# Autodesk Inventor assembly: Assembly1
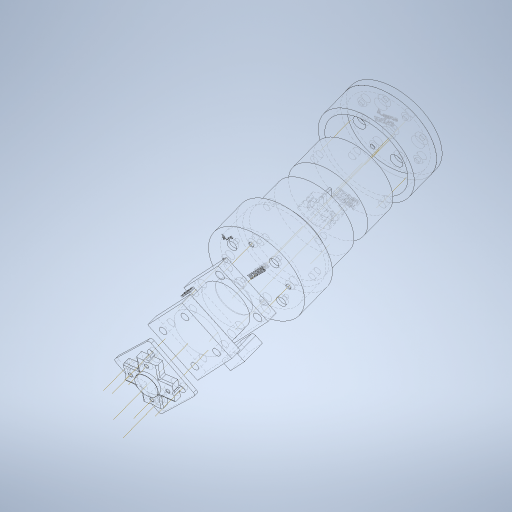
[picture p0: Inventor's stored thumbnail of the model, 512x512]
Saved by Autodesk Inventor 2024 (Build 280153000, 153)
## iProperties
Created: 2024-08-06
Part Number: Assembly1
Document SubType Name: Assembly
Designer: maint
Author: maint
## Documents named in this file (8)
- G:\3dprintings\Assembly1.iam
- G:\3dprintings\adapter_final2.ipt
- G:\3dprintings\adaptor_spine_transducer_names.ipt
- G:\3dprintings\adaptor_spine_base_names.ipt
- C:\Users\maint\Downloads\91292A770_18-8 Stainless Steel Socket Head Screw\91292A770_18-8 Stainless Steel Socket Head Screw.iam
- C:\Users\maint\Downloads\91263A913_Zinc-Plated Alloy Steel Hex Drive Flat Head Screw\91263A913_Zinc-Plated Alloy Steel Hex Drive Flat Head Screw.iam
- G:\3dprintings\spine.ipt
- G:\3dprintings\sensor_AMTI.ipt
## Components (17 placed, 7 different names)
1. adapter_final2:2 — Flush:2, Mate:3, Mate:5, Mate:9, Mate:11, Mate:14, Mate:16, Mate:20, Mate:21, Mate:24
2. adaptor_spine_transducer_names:1 — Flush:1, Flush:2, Mate:29, Mate:30, Mate:32, Mate:33, Mate:34, Mate:43, Mate:52
3. adaptor_spine_base_names:1 — Flush:1, Mate:26, Mate:45, Mate:46, Mate:47, Mate:48, Mate:57, Mate:58
4. 91292A770_18-8 Stainless Steel Socket Head Screw:1 [sub-assembly] — Mate:12
5. 91292A770_18-8 Stainless Steel Socket Head Screw:2 [sub-assembly] — Mate:2
6. 91292A770_18-8 Stainless Steel Socket Head Screw:3 [sub-assembly] — Mate:8, Mate:10
7. 91292A770_18-8 Stainless Steel Socket Head Screw:4 [sub-assembly] — Mate:6, Mate:7
8. 91263A913_Zinc-Plated Alloy Steel Hex Drive Flat Head Screw:1 [sub-assembly] — Mate:13, Mate:15
9. 91263A913_Zinc-Plated Alloy Steel Hex Drive Flat Head Screw:2 [sub-assembly] — Mate:17
10. 91263A913_Zinc-Plated Alloy Steel Hex Drive Flat Head Screw:3 [sub-assembly] — Mate:19
11. 91263A913_Zinc-Plated Alloy Steel Hex Drive Flat Head Screw:4 [sub-assembly] — Mate:18
12. 91292A770_18-8 Stainless Steel Socket Head Screw:5 [sub-assembly] — Mate:31
13. 91292A770_18-8 Stainless Steel Socket Head Screw:6 [sub-assembly] — Mate:36, Mate:37
14. 91292A770_18-8 Stainless Steel Socket Head Screw:7 [sub-assembly] — Mate:38
15. 91292A770_18-8 Stainless Steel Socket Head Screw:8 [sub-assembly] — Mate:40, Mate:41
16. spine:1 — Mate:42, Mate:43, Mate:44, Mate:49, Mate:50, Mate:57
17. sensor_AMTI:1 — Mate:51, Mate:54, Mate:55
## Relationships (57: Mate 55, Flush 2)
- Flush:1 (-203.2 mm): adaptor_spine_transducer_names:1 ↔ adaptor_spine_base_names:1
- Flush:2 (203.2 mm): adapter_final2:2 ↔ adaptor_spine_transducer_names:1
- Mate:2: 91292A770_18-8 Stainless Steel Socket Head Screw:2
- Mate:3: adapter_final2:2
- Mate:4
- Mate:5: adapter_final2:2
- Mate:6: 91292A770_18-8 Stainless Steel Socket Head Screw:4
- Mate:7: 91292A770_18-8 Stainless Steel Socket Head Screw:4
- Mate:8: 91292A770_18-8 Stainless Steel Socket Head Screw:3
- Mate:9: adapter_final2:2
- Mate:10: 91292A770_18-8 Stainless Steel Socket Head Screw:3
- Mate:11: adapter_final2:2
- Mate:12: 91292A770_18-8 Stainless Steel Socket Head Screw:1
- Mate:13: 91263A913_Zinc-Plated Alloy Steel Hex Drive Flat Head Screw:1
- Mate:14: adapter_final2:2
- Mate:15: 91263A913_Zinc-Plated Alloy Steel Hex Drive Flat Head Screw:1
- Mate:16: adapter_final2:2
- Mate:17: 91263A913_Zinc-Plated Alloy Steel Hex Drive Flat Head Screw:2
- Mate:18: 91263A913_Zinc-Plated Alloy Steel Hex Drive Flat Head Screw:4
- Mate:19: 91263A913_Zinc-Plated Alloy Steel Hex Drive Flat Head Screw:3
- Mate:20: adapter_final2:2
- Mate:21: adapter_final2:2
- Mate:22
- Mate:23
- Mate:24: adapter_final2:2
- Mate:26: adaptor_spine_base_names:1
- Mate:28
- Mate:29: adaptor_spine_transducer_names:1
- Mate:30: adaptor_spine_transducer_names:1
- Mate:31: 91292A770_18-8 Stainless Steel Socket Head Screw:5
- Mate:32: adaptor_spine_transducer_names:1
- Mate:33: adaptor_spine_transducer_names:1
- Mate:34: adaptor_spine_transducer_names:1
- Mate:35
- Mate:36: 91292A770_18-8 Stainless Steel Socket Head Screw:6
- Mate:37: 91292A770_18-8 Stainless Steel Socket Head Screw:6
- Mate:38: 91292A770_18-8 Stainless Steel Socket Head Screw:7
- Mate:39
- Mate:40: 91292A770_18-8 Stainless Steel Socket Head Screw:8
- Mate:41: 91292A770_18-8 Stainless Steel Socket Head Screw:8
- Mate:42: spine:1
- Mate:43: adaptor_spine_transducer_names:1 ↔ spine:1
- Mate:44: spine:1
- Mate:45: adaptor_spine_base_names:1
- Mate:46: adaptor_spine_base_names:1
- Mate:47: adaptor_spine_base_names:1
- Mate:48: adaptor_spine_base_names:1
- Mate:49: spine:1
- Mate:50: spine:1
- Mate:51: sensor_AMTI:1
- Mate:52: adaptor_spine_transducer_names:1
- Mate:53
- Mate:54: sensor_AMTI:1
- Mate:55: sensor_AMTI:1
- Mate:56
- Mate:57: adaptor_spine_base_names:1 ↔ spine:1
- Mate:58: adaptor_spine_base_names:1
## Named parameters: Finish10_Area = 0, Finish10_Thickness = 0.05 mm, Finish11_Area = 406.483, Finish11_Thickness = 0.05 mm, Finish12_Area = 109.98, Finish13_Area = 200.638, Finish1_Area = 118.41, Finish2_Area = 81.1285, Finish3_Area = 57.7347, Finish4_Area = 0, Finish4_Thickness = 0.05 mm, Finish5_Area = 0, Finish5_Thickness = 0.05 mm, Finish6_Area = 0, Finish6_Thickness = 0.05 mm, Finish7_Area = 0, Finish7_Thickness = 0.05 mm, Finish8_Area = 0, Finish8_Thickness = 0.05 mm, Finish9_Area = 0, Finish9_Thickness = 0.05 mm
note: some values were not read from the file. Shown as the stored number, unit unknown: "Finish10_Area", "Finish11_Area", "Finish12_Area", "Finish13_Area", "Finish1_Area", "Finish2_Area", "Finish3_Area", "Finish4_Area", "Finish5_Area", "Finish6_Area", "Finish7_Area", "Finish8_Area", "Finish9_Area".
